# Autodesk Inventor assembly: 20X20 lift conecter with 20X20.ipt
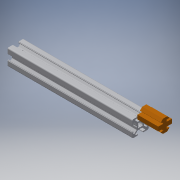
[picture p0: Inventor's stored thumbnail of the model, 180x180]
Saved by Autodesk Inventor 2019 (Build 230136000, 136)
## iProperties
Created: 2018-10-25
Part Number: 20X20 lift conecter with 20X20.ipt
Document SubType Name: Assembly
Designer: User
Author: User
## Documents named in this file (3)
- C:\Robotics\CAD\2018-19_CAD\Collection\20X20 lift conecter with 20X20.ipt.iam
- C:\Robotics\CAD\2018-19_CAD\Collection\20X20 lift conecter.ipt
- C:\Robotics\CAD\COTSParts\Bosch Extrusion\Bosch 20x20 6 in.ipt
## Components (2 placed, 2 different names)
1. 20X20 lift conecter:1 — Mate:1, Angle:1
2. Bosch 20x20 6 in:1 — Mate:1, Angle:1
## Relationships (2: Mate 1, Angle 1)
- Mate:1: 20X20 lift conecter:1 ↔ Bosch 20x20 6 in:1
- Angle:1 (0 deg): 20X20 lift conecter:1 ↔ Bosch 20x20 6 in:1
